# Autodesk Inventor assembly: BoomWithConnector
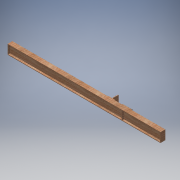
[picture p0: Inventor's stored thumbnail of the model, 180x180]
Saved by Autodesk Inventor 2016 SP1 (Build 200210100, 210)
## iProperties
Created: 2016-04-01
Part Number: BoomWithConnector
Document SubType Name: Assembly
Designer: mkepler
Author: mkepler
## Documents named in this file (3)
- C:\Users\Wes\Documents\School Stuff\ECE 499\ece-499-hw1\design\mechanical\Boom\BoomWithConnector.iam
- C:\Users\Wes\Documents\School Stuff\ECE 499\ece-499-hw1\design\mechanical\Shaft\RotatorTop.ipt
- C:\Users\Wes\Documents\School Stuff\ECE 499\ece-499-hw1\design\mechanical\Boom\Boom.ipt
## Components (2 placed, 2 different names)
1. RotatorTop:1 — Mate:1, Mate:2, Mate:3, Mate:4
2. Boom:1 — Mate:1, Mate:2, Mate:3, Mate:4
## Relationships (4: Mate 4)
- Mate:1: RotatorTop:1 ↔ Boom:1
- Mate:2 (2 mm): RotatorTop:1 ↔ Boom:1
- Mate:3 (2 mm): RotatorTop:1 ↔ Boom:1
- Mate:4: RotatorTop:1 ↔ Boom:1
